# Autodesk Inventor assembly: 60pc_keey_v1.1
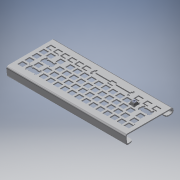
[picture p0: Inventor's stored thumbnail of the model, 180x180]
Saved by Autodesk Inventor 2018 (Build 220112000, 112)
## iProperties
Created: 2018-02-17
Part Number: 60pc_keey_v1.1
Document SubType Name: Assembly
Designer: ConnorDevitt
Author: ConnorDevitt
## Documents named in this file (3)
- C:\Users\ConnorDevitt.MSI\Documents\Keyboard\60pc_Keeb\HW\Mech\Small_FormFactor(v1.1)\60pc_keey_v1.1.iam
- C:\Users\ConnorDevitt.MSI\Documents\Keyboard\60pc_Keeb\HW\Mech\Small_FormFactor(v1.1)\Frame_v1.1.ipt
- C:\Users\ConnorDevitt.MSI\Documents\Keyboard\60pc_Keeb\HW\Mech\MX .ipt
## Components (2 placed, 2 different names)
1. Frame_v1.1:1 — Insert:1
2. MX :1 — Insert:1
## Relationships (1: Insert 1)
- Insert:1: Frame_v1.1:1 ↔ MX :1
